# Autodesk Inventor assembly: ASY GBK 2210 short wall shield 4
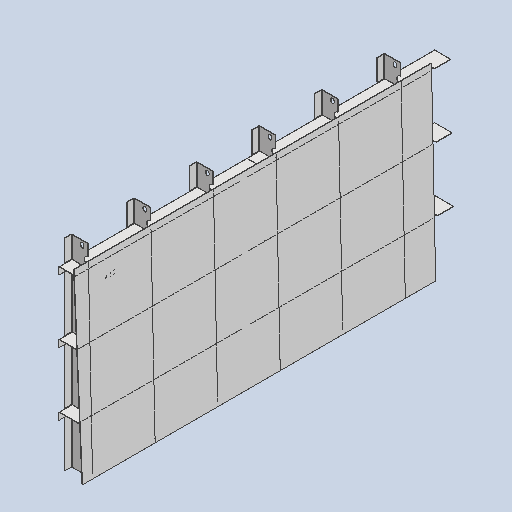
[picture p0: Inventor's stored thumbnail of the model, 512x512]
Saved by Autodesk Inventor 2026.3 (Build 303398000, 398)
## iProperties
Created: 2026-05-07
Part Number: ASY GBK 2210 short wall shield 4
Document SubType Name: Assembly
Designer: pokla
Stock Number: 2210
Mass: 252568 g
Surface Area: 163192 cm^2
Volume: 32174.3 cm^3
Density: 7.85 g/cm^3
Author: admin
Comments: поменял
## Documents named in this file (7)
- C:\Users\admin\Documents\Inventor\GBK-Gubkinskiy\ASY GBK 2210 short wall shield 4.iam
- C:\Users\admin\Documents\Inventor\GBK-Gubkinskiy\GBK 0101 main rib.ipt
- C:\Users\admin\Documents\Inventor\GBK-Gubkinskiy\GBK 2211 shield 4.ipt
- C:\Users\admin\Documents\Inventor\GBK-Gubkinskiy\GBK 0202 stringer 4.ipt
- C:\Users\admin\Documents\Inventor\GBK-Gubkinskiy\GBK 0203 stringer 5.ipt
- C:\Users\admin\Documents\Inventor\GBK-Gubkinskiy\GBK 0204 stringer 6.ipt
- C:\Users\admin\Documents\Inventor\GBK-Gubkinskiy\GBK 0201 second rib.ipt
## Components (13 placed, 5 different names)
1. GBK 0202 stringer 4:1 — Rigid:6, Rigid:1
2. GBK 0202 stringer 4:2 — Rigid:1
3. GBK 0203 stringer 5:1 — Rigid:5, Rigid:2
4. GBK 0203 stringer 5:2 — Rigid:2
5. GBK 0204 stringer 6:1 — Rigid:4, Rigid:3, Flush:1
6. GBK 0204 stringer 6:2 — Rigid:3, Flush:2
7. GBK 2211 shield 4:1 — Mate:3, Flush:2, Mate:4
8. GBK 0201 second rib:1 — Rigid:6, Rigid:5, Rigid:4, Mate:1, Mate:2, Mate:3
9. GBK 0201 second rib:2
10. GBK 0201 second rib:3
11. GBK 0201 second rib:4
12. GBK 0201 second rib:5
13. GBK 0201 second rib:6
## Component patterns: (6 elements, first: GBK 0201 second rib:1)
## Relationships (12: WeldJoint 6, Mate 4, Flush 2)
- Rigid:6 [WeldJoint] (4 mm): GBK 0202 stringer 4:1 ↔ GBK 0201 second rib:1
- Rigid:1 [WeldJoint] (1 mm): GBK 0202 stringer 4:1 ↔ GBK 0202 stringer 4:2
- Rigid:5 [WeldJoint] (4 mm): GBK 0203 stringer 5:1 ↔ GBK 0201 second rib:1
- Rigid:2 [WeldJoint] (1 mm): GBK 0203 stringer 5:1 ↔ GBK 0203 stringer 5:2
- Rigid:4 [WeldJoint] (4 mm): GBK 0204 stringer 6:1 ↔ GBK 0201 second rib:1
- Rigid:3 [WeldJoint] (1 mm): GBK 0204 stringer 6:1 ↔ GBK 0204 stringer 6:2
- Mate:1: GBK 0201 second rib:1
- Flush:1: GBK 0204 stringer 6:1
- Mate:2: GBK 0201 second rib:1
- Mate:3: GBK 2211 shield 4:1 ↔ GBK 0201 second rib:1
- Flush:2 (155 mm): GBK 0204 stringer 6:2 ↔ GBK 2211 shield 4:1
- Mate:4: GBK 2211 shield 4:1
## Named parameters: основание_длина_нижнего = 200 mm, основание_длина_верхнего = 100 mm, стрингер_глубина_1 = 190.70056 mm, стрингер_глубина_2 = 179.35977 mm, стрингер_глубина_3 = 168.01899 mm, стрингер_глубина_4 = 156.6782 mm, стрингер_глубина_5 = 145.33742 mm, стрингер_глубина_6 = 133.99663 mm, стрингер_глубина_7 = 122.65585 mm, стрингер_глубина_8 = 111.31507 mm, Лист_ширина = 1480 mm, ребро_усилителей = 60 mm, паз_под_стрингер_глубина = 70 mm, паз_под_стрингер_толщина = 5 mm, отступ_от_пола_до_первого_стрингера = 410 mm, шаг_стрингеров = 500 mm, радиус_выреза_под_сварку = 30 mm, нахлест_шпангоутов_1_2 = 150 mm, нахлест_шпангоутов_2_3 = 120 mm, Стрингер_длина = 1489.5 mm, Лист_длина = 2980 mm, Шаг_шпангоутов = 496.66667 mm
